# Autodesk Inventor assembly: TI-83x
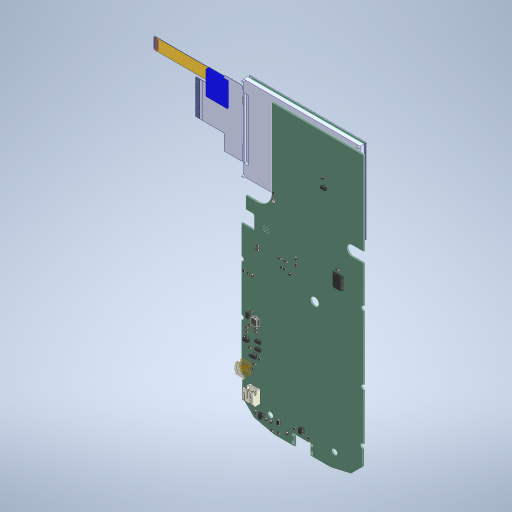
[picture p0: Inventor's stored thumbnail of the model, 512x512]
Saved by Autodesk Inventor 2023 (Build 270158000, 158)
## iProperties
Created: 2023-03-09
Part Number: TI-83x
Document SubType Name: Assembly
Designer: Peter
Title: TI-83x
Author: Peter
## Documents named in this file (3)
- D:\Documents\KiCad\6.0\projects\TI-83x\CAD\TI-83x.iam
- D:\Documents\KiCad\6.0\projects\TI-83x\CAD\TI-83x.ipt
- D:\Documents\KiCad\6.0\projects\TI-83x\CAD\NHD-2.8-240320AF-CSXP-F-CTP.ipt
## Components (2 placed, 2 different names)
1. TI-83x_PCB:1 — Mate:1, Angle:1, Mate:2
2. NHD-2.8-240320AF-CSXP-F-CTP:1 — Mate:1, Angle:1, Mate:2
## Relationships (3: Mate 2, Angle 1)
- Mate:1: TI-83x_PCB:1 ↔ NHD-2.8-240320AF-CSXP-F-CTP:1
- Angle:1 (0 deg): TI-83x_PCB:1 ↔ NHD-2.8-240320AF-CSXP-F-CTP:1
- Mate:2: TI-83x_PCB:1 ↔ NHD-2.8-240320AF-CSXP-F-CTP:1
